# Autodesk Inventor assembly: a shock strut
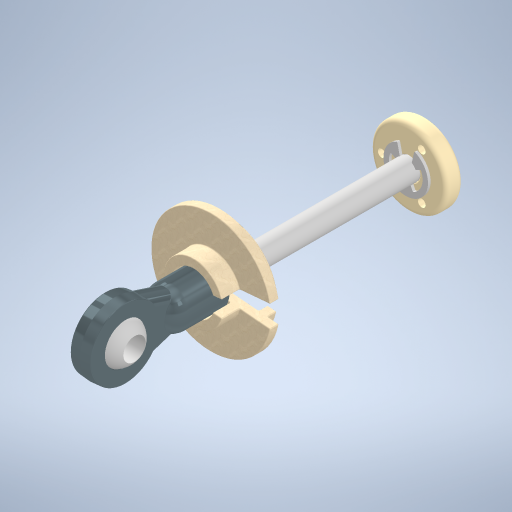
[picture p0: Inventor's stored thumbnail of the model, 512x512]
Saved by Autodesk Inventor 2024 (Build 280153000, 153)
## iProperties
Created: 2023-07-07
Part Number: a shock strut
Document SubType Name: Assembly
Designer: birud
Author: birud
## Documents named in this file (6)
- C:\Users\birud\OneDrive\Desktop\Openers\a shock strut.iam
- C:\Users\birud\OneDrive\Desktop\Openers\Piston-1.ipt
- C:\Users\birud\OneDrive\Desktop\Openers\shock shaft-1.ipt
- C:\Users\birud\OneDrive\Desktop\Openers\SA E-Clip.ipt
- C:\Users\birud\OneDrive\Desktop\Openers\a ball end.iam
- C:\Users\birud\OneDrive\Desktop\Openers\SA Spring Cup.ipt
## Components (6 placed, 5 different names)
1. Piston-1:1 — Mate:1, Mate:3, Flush:1, Mate:5
2. shock shaft-1:1 — Mate:1, Mate:2, Flush:1, Mate:4, Mate:6, Mate:7, Mate:8
3. SA E-Clip:1 — Mate:2, Mate:3
4. SA E-Clip:2 — Mate:4, Mate:5
5. a ball end:1 [sub-assembly] — Mate:6, Mate:7, Mate:9
6. SA Spring Cup:1 — Mate:8, Mate:9
## Relationships (10: Mate 9, Flush 1)
- Mate:1: Piston-1:1 ↔ shock shaft-1:1
- Mate:2: shock shaft-1:1 ↔ SA E-Clip:1
- Mate:3: Piston-1:1 ↔ SA E-Clip:1
- Flush:1: Piston-1:1 ↔ shock shaft-1:1
- Mate:4: shock shaft-1:1 ↔ SA E-Clip:2
- Mate:5: Piston-1:1 ↔ SA E-Clip:2
- Mate:6: shock shaft-1:1 ↔ a ball end:1
- Mate:7: shock shaft-1:1 ↔ a ball end:1
- Mate:8: shock shaft-1:1 ↔ SA Spring Cup:1
- Mate:9: a ball end:1 ↔ SA Spring Cup:1
